# Autodesk Inventor assembly: Maccaronikanone
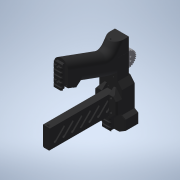
[picture p0: Inventor's stored thumbnail of the model, 180x180]
Saved by Autodesk Inventor 2021 (Build 250183000, 183)
## iProperties
Created: 2021-03-07
Part Number: Maccaronikanone
Document SubType Name: Assembly
Designer: Lukas
Author: Lukas
## Documents named in this file (26)
- Z:\Datastorrage\Projects\Maccaroni-Gun\Inventor files\Maccaronikanone.iam
- Z:\Datastorrage\Projects\Maccaroni-Gun\Inventor files\Maccaroni.ipt
- Z:\Datastorrage\Projects\Maccaroni-Gun\Inventor files\Motor_18mm.ipt
- Z:\Datastorrage\Projects\Maccaroni-Gun\Inventor files\Motor_holder.ipt
- Z:\Datastorrage\Projects\Maccaroni-Gun\Inventor files\Antriebsrad.ipt
- Z:\Datastorrage\Projects\Maccaroni-Gun\Inventor files\Abzugsgehäuse.ipt
- Z:\Datastorrage\Projects\Maccaroni-Gun\Inventor files\Magazin_Boden.ipt
- Z:\Datastorrage\Projects\Maccaroni-Gun\Inventor files\Griff.ipt
- Z:\Datastorrage\Projects\Maccaroni-Gun\Inventor files\Hammer_Halter.ipt
- Z:\Datastorrage\Projects\Maccaroni-Gun\Inventor files\Hammer2.ipt
- Z:\Datastorrage\Projects\Maccaroni-Gun\Inventor files\Top_Lid.ipt
- Z:\Datastorrage\Projects\Maccaroni-Gun\Inventor files\Stiftleiste_3Pin.ipt
- Z:\Datastorrage\Projects\Maccaroni-Gun\Inventor files\Stiftleiste_Halter.ipt
- Z:\Datastorrage\Projects\Maccaroni-Gun\Inventor files\ESC_Halter.ipt
- Z:\Datastorrage\Projects\Maccaroni-Gun\Inventor files\Hauptschalter.ipt
- Z:\Datastorrage\Projects\Maccaroni-Gun\Inventor files\Ladesteckerhalter.ipt
- Z:\Datastorrage\Projects\Maccaroni-Gun\Inventor files\Deckel.ipt
- Z:\Datastorrage\Projects\Maccaroni-Gun\Inventor files\Underrail.ipt
- Z:\Datastorrage\Projects\Maccaroni-Gun\Inventor files\Picatinny Rail.ipt
- Z:\Datastorrage\Projects\Maccaroni-Gun\Inventor files\Picatinny Rail short.ipt
- Z:\Datastorrage\Projects\Maccaroni-Gun\Inventor files\Magazin2.ipt
- Z:\Datastorrage\Projects\Maccaroni-Gun\Inventor files\Magazin2_Stössel.ipt
- Z:\Datastorrage\Projects\Maccaroni-Gun\Inventor files\ML2204B 2204-260kv.ipt
- Z:\Datastorrage\Projects\Maccaroni-Gun\Inventor files\Pinion.ipt
- Z:\Datastorrage\Projects\Maccaroni-Gun\Inventor files\XXX.XXXXPCB_Assy_Revision_Driveunit_RS485.ipt
- Z:\Datastorrage\Projects\Maccaroni-Gun\Inventor files\Motor_mount.ipt
## Components (29 placed, 25 different names)
1. Abzugsgehäuse:1 — Flush:1, Flush:2, Flush:3, Mate:61, Mate:62, Angle:1, Angle:2, Mate:70, Mate:76, Mate:82, Mate:83, Mate:84, Flush:10, Mate:93, Mate:98, Mate:99, Flush:11, Flush:12, Mate:102, Mate:103, Flush:13, Flush:14, Mate:104, Mate:105, Flush:16, Mate:127, Mate:128, Mate:129, Mate:139, Mate:140, Mate:161, Mate:162, Mate:164
2. Maccaroni:1 — Mate:63, Mate:70
3. Motor_holder:1 — Mate:55, Mate:56, Mate:57, Mate:58, Mate:59, Mate:60, Mate:61, Mate:62, Angle:1
4. Motor_18mm:1 — Mate:58, Mate:59, Mate:60, Insert:2, Mate:64
5. Motor_18mm:2 — Mate:55, Mate:56, Mate:57, Insert:1, Mate:65
6. Antriebsrad:1 — Insert:1, Mate:65
7. Antriebsrad:2 — Insert:2, Mate:64
8. Magazin2:1 — Angle:2, Mate:139, Mate:140, Flush:18, Flush:19, Mate:141, Mate:142, Mate:143
9. Magazin_Boden:1 — Flush:18, Flush:19, Mate:141
10. Griff:1 — Mate:76, Mate:91, Mate:93, Mate:117, Mate:118, Mate:161
11. Hammer_Halter:1 — Mate:82, Mate:83, Mate:84, Mate:87, Angle:3
12. Hammer2:1 — Mate:87, Angle:3
13. Top_Lid:1 — Mate:91, Flush:10, Mate:107, Mate:124, Mate:125, Mate:126, Flush:17
14. Stiftleiste_Halter:1 — Mate:103, Flush:13, Mate:105, Mate:106
15. Stiftleiste_Halter:2 — Mate:102, Flush:14, Mate:104, Flush:15
16. Stiftleiste_3Pin:1 — Mate:99, Flush:11, Mate:106
17. Stiftleiste_3Pin:2 — Mate:98, Flush:12, Flush:15
18. ESC_Halter:1 — Mate:107, Mate:124, Mate:125
19. Hauptschalter:1 — Mate:117, Mate:118, Mate:119, Mate:120, Mate:121
20. Ladesteckerhalter:1 — Mate:119, Mate:120, Mate:121, Mate:137, Mate:138
21. Deckel:1 — Mate:126, Flush:16, Flush:17, Mate:132, Mate:133, Mate:136
22. Underrail:1 — Mate:127, Mate:128, Mate:129
23. Picatinny Rail:1 — Mate:132, Mate:133, Mate:136
24. Picatinny Rail short:1 — Mate:137, Mate:138
25. Magazin2_Stössel:1 — Mate:142, Mate:143
26. ML2204B 2204-260kv:1 — Mate:153, Mate:154, Mate:168, Mate:169, Angle:4, Angle:5
27. Pinion:1 — Mate:153, Mate:154, Angle:5
28. XXX.XXXXPCB_Assy_Revision_Driveunit_RS485:1 — Mate:165, Mate:166, Mate:167
29. Motor_mount:1 — Mate:162, Mate:164, Mate:165, Mate:166, Mate:167, Mate:168, Mate:169, Angle:4
## Relationships (80: Mate 60, Flush 13, Angle 5, Insert 2)
- Flush:1: Abzugsgehäuse:1
- Flush:2: Abzugsgehäuse:1
- Flush:3: Abzugsgehäuse:1
- Mate:55: Motor_holder:1 ↔ Motor_18mm:2
- Mate:56: Motor_holder:1 ↔ Motor_18mm:2
- Mate:57: Motor_holder:1 ↔ Motor_18mm:2
- Mate:58: Motor_holder:1 ↔ Motor_18mm:1
- Mate:59: Motor_holder:1 ↔ Motor_18mm:1
- Mate:60: Motor_holder:1 ↔ Motor_18mm:1
- Mate:61: Abzugsgehäuse:1 ↔ Motor_holder:1
- Mate:62: Abzugsgehäuse:1 ↔ Motor_holder:1
- Angle:1 (0 deg): Abzugsgehäuse:1 ↔ Motor_holder:1
- Mate:63: Maccaroni:1
- Insert:1: Motor_18mm:2 ↔ Antriebsrad:1
- Insert:2: Motor_18mm:1 ↔ Antriebsrad:2
- Mate:64: Motor_18mm:1 ↔ Antriebsrad:2
- Mate:65: Motor_18mm:2 ↔ Antriebsrad:1
- Angle:2 (180 deg): Abzugsgehäuse:1 ↔ Magazin2:1
- Mate:70 (13 mm): Abzugsgehäuse:1 ↔ Maccaroni:1
- [Mate]: Maccaroni:1 ↔ Magazin2:1
- [Mate]: Abzugsgehäuse:1 ↔ Magazin2:1
- Mate:76: Abzugsgehäuse:1 ↔ Griff:1
- Mate:82: Abzugsgehäuse:1 ↔ Hammer_Halter:1
- Mate:83: Abzugsgehäuse:1 ↔ Hammer_Halter:1
- Mate:84: Abzugsgehäuse:1 ↔ Hammer_Halter:1
- Mate:87: Hammer_Halter:1 ↔ Hammer2:1
- Angle:3 (0 deg): Hammer_Halter:1 ↔ Hammer2:1
- Mate:91 (0.2 mm): Griff:1 ↔ Top_Lid:1
- Flush:10: Abzugsgehäuse:1 ↔ Top_Lid:1
- Mate:93: Abzugsgehäuse:1 ↔ Griff:1
- Mate:98: Abzugsgehäuse:1 ↔ Stiftleiste_3Pin:2
- Mate:99: Abzugsgehäuse:1 ↔ Stiftleiste_3Pin:1
- Flush:11: Abzugsgehäuse:1 ↔ Stiftleiste_3Pin:1
- Flush:12: Abzugsgehäuse:1 ↔ Stiftleiste_3Pin:2
- Mate:102 (0.2 mm): Abzugsgehäuse:1 ↔ Stiftleiste_Halter:2
- Mate:103 (0.2 mm): Abzugsgehäuse:1 ↔ Stiftleiste_Halter:1
- Flush:13: Abzugsgehäuse:1 ↔ Stiftleiste_Halter:1
- Flush:14: Abzugsgehäuse:1 ↔ Stiftleiste_Halter:2
- Mate:104: Abzugsgehäuse:1 ↔ Stiftleiste_Halter:2
- Mate:105: Abzugsgehäuse:1 ↔ Stiftleiste_Halter:1
- Mate:106: Stiftleiste_Halter:1 ↔ Stiftleiste_3Pin:1
- Flush:15: Stiftleiste_Halter:2 ↔ Stiftleiste_3Pin:2
- Mate:107: Top_Lid:1 ↔ ESC_Halter:1
- Mate:117: Griff:1 ↔ Hauptschalter:1
- Mate:118: Griff:1 ↔ Hauptschalter:1
- Mate:119: Hauptschalter:1 ↔ Ladesteckerhalter:1
- Mate:120: Hauptschalter:1 ↔ Ladesteckerhalter:1
- Mate:121 (10.9 mm): Hauptschalter:1 ↔ Ladesteckerhalter:1
- Mate:124: Top_Lid:1 ↔ ESC_Halter:1
- Mate:125: Top_Lid:1 ↔ ESC_Halter:1
- Mate:126: Top_Lid:1 ↔ Deckel:1
- Flush:16: Abzugsgehäuse:1 ↔ Deckel:1
- Flush:17: Top_Lid:1 ↔ Deckel:1
- Mate:127: Abzugsgehäuse:1 ↔ Underrail:1
- Mate:128: Abzugsgehäuse:1 ↔ Underrail:1
- Mate:129: Abzugsgehäuse:1 ↔ Underrail:1
- Mate:132: Deckel:1 ↔ Picatinny Rail:1
- Mate:133: Deckel:1 ↔ Picatinny Rail:1
- Mate:136: Deckel:1 ↔ Picatinny Rail:1
- Mate:137: Ladesteckerhalter:1 ↔ Picatinny Rail short:1
- Mate:138: Ladesteckerhalter:1 ↔ Picatinny Rail short:1
- Mate:139 (0.1 mm): Abzugsgehäuse:1 ↔ Magazin2:1
- Mate:140 (0.1 mm): Abzugsgehäuse:1 ↔ Magazin2:1
- Flush:18: Magazin2:1 ↔ Magazin_Boden:1
- Flush:19: Magazin2:1 ↔ Magazin_Boden:1
- Mate:141: Magazin2:1 ↔ Magazin_Boden:1
- Mate:142 (0.15 mm): Magazin2:1 ↔ Magazin2_Stössel:1
- Mate:143 (0.15 mm): Magazin2:1 ↔ Magazin2_Stössel:1
- Mate:153: ML2204B 2204-260kv:1 ↔ Pinion:1
- Mate:154: ML2204B 2204-260kv:1 ↔ Pinion:1
- Mate:161: Abzugsgehäuse:1 ↔ Griff:1
- Mate:162: Abzugsgehäuse:1 ↔ Motor_mount:1
- Mate:164: Abzugsgehäuse:1 ↔ Motor_mount:1
- Mate:165: XXX.XXXXPCB_Assy_Revision_Driveunit_RS485:1 ↔ Motor_mount:1
- Mate:166: XXX.XXXXPCB_Assy_Revision_Driveunit_RS485:1 ↔ Motor_mount:1
- Mate:167: XXX.XXXXPCB_Assy_Revision_Driveunit_RS485:1 ↔ Motor_mount:1
- Mate:168: ML2204B 2204-260kv:1 ↔ Motor_mount:1
- Mate:169: ML2204B 2204-260kv:1 ↔ Motor_mount:1
- Angle:4 (0 deg): ML2204B 2204-260kv:1 ↔ Motor_mount:1
- Angle:5 (0 deg): ML2204B 2204-260kv:1 ↔ Pinion:1
